# Autodesk Inventor assembly: Montagem Válvula Borboleta
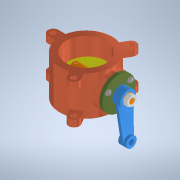
[picture p0: Inventor's stored thumbnail of the model, 180x180]
Saved by Autodesk Inventor 2021 (Build 250183000, 183)
## iProperties
Created: 2021-04-23
Part Number: Montagem Válvula Borboleta
Document SubType Name: Assembly
Designer: rubia
Author: rubia
## Documents named in this file (9)
- C:\Users\rubia\OneDrive\Documentos\Inventor\Rubia_ASR6\Montagem Válvula Borboleta.iam
- C:\Users\rubia\OneDrive\Documentos\Inventor\Rubia_ASR6\Corpo da Valvula.ipt
- C:\Users\rubia\OneDrive\Documentos\Inventor\Rubia_ASR6\Retentor.ipt
- C:\Users\rubia\OneDrive\Documentos\Inventor\Rubia_ASR6\Parafuso.ipt
- C:\Users\rubia\OneDrive\Documentos\Inventor\Rubia_ASR6\Eixo.ipt
- C:\Users\rubia\OneDrive\Documentos\Inventor\Rubia_ASR6\Manipulo.ipt
- C:\Users\rubia\OneDrive\Documentos\Inventor\Rubia_ASR6\Placa.ipt
- C:\Users\rubia\OneDrive\Documentos\Inventor\Rubia_ASR6\Pino.ipt
- C:\Users\rubia\OneDrive\Documentos\Inventor\Rubia_ASR6\Porca.ipt
## Components (11 placed, 8 different names)
1. Corpo da Valvula:1 — Coincidente:1, Coincidente:2, Coincidente:3, Coincidente:4, Coincidente:11, Coincidente:12
2. Retentor:1 — Coincidente:1, Coincidente:2, Coincidente:3, Coincidente:4, Coincidente:5, Coincidente:6, Coincidente:7, Coincidente:8, Coincidente:9, Coincidente:10, Coincidente:24
3. Parafuso:1 — Coincidente:8, Coincidente:10
4. Parafuso:2 — Coincidente:7, Coincidente:9
5. Parafuso:3 — Coincidente:5, Coincidente:6
6. Eixo:1 — Coincidente:11, Coincidente:12, Coincidente:13, Coincidente:14, Coincidente:16, Coincidente:17, Coincidente:18, Coincidente:21, Coincidente:22
7. Manipulo:1 — Coincidente:13, Coincidente:14, Coincidente:23, Coincidente:24
8. Placa:1 — Coincidente:16, Coincidente:17, Coincidente:18, Coincidente:19, Alinhado:1, Coincidente:20, Alinhado:2
9. Pino:1 — Coincidente:19, Alinhado:1
10. Pino:2 — Coincidente:20, Alinhado:2
11. Porca:1 — Coincidente:21, Coincidente:22, Coincidente:23
## Relationships (25: Mate 23, Flush 2)
- Coincidente:1 [Mate]: Corpo da Valvula:1 ↔ Retentor:1
- Coincidente:2 [Mate]: Corpo da Valvula:1 ↔ Retentor:1
- Coincidente:3 [Mate]: Corpo da Valvula:1 ↔ Retentor:1
- Coincidente:4 [Mate]: Corpo da Valvula:1 ↔ Retentor:1
- Coincidente:5 [Mate]: Retentor:1 ↔ Parafuso:3
- Coincidente:6 [Mate]: Retentor:1 ↔ Parafuso:3
- Coincidente:7 [Mate]: Retentor:1 ↔ Parafuso:2
- Coincidente:8 [Mate]: Retentor:1 ↔ Parafuso:1
- Coincidente:9 [Mate]: Retentor:1 ↔ Parafuso:2
- Coincidente:10 [Mate]: Retentor:1 ↔ Parafuso:1
- Coincidente:11 [Mate]: Corpo da Valvula:1 ↔ Eixo:1
- Coincidente:12 [Mate]: Corpo da Valvula:1 ↔ Eixo:1
- Coincidente:13 [Mate]: Eixo:1 ↔ Manipulo:1
- Coincidente:14 [Mate]: Eixo:1 ↔ Manipulo:1
- Coincidente:16 [Mate]: Eixo:1 ↔ Placa:1
- Coincidente:17 [Mate]: Eixo:1 ↔ Placa:1
- Coincidente:18 [Mate]: Eixo:1 ↔ Placa:1
- Coincidente:19 [Mate]: Placa:1 ↔ Pino:1
- Alinhado:1 [Flush]: Placa:1 ↔ Pino:1
- Coincidente:20 [Mate]: Placa:1 ↔ Pino:2
- Alinhado:2 [Flush]: Placa:1 ↔ Pino:2
- Coincidente:21 [Mate]: Eixo:1 ↔ Porca:1
- Coincidente:22 [Mate]: Eixo:1 ↔ Porca:1
- Coincidente:23 [Mate]: Manipulo:1 ↔ Porca:1
- Coincidente:24 [Mate] (2 mm): Retentor:1 ↔ Manipulo:1
